# Autodesk Inventor assembly: Final Assembly
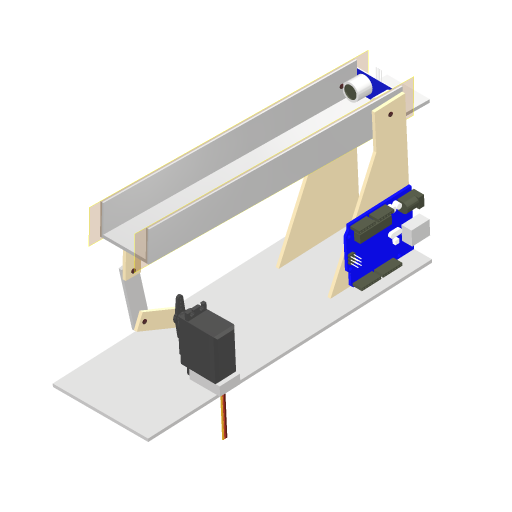
[picture p0: Inventor's stored thumbnail of the model, 512x512]
Saved by Autodesk Inventor 2024 (Build 280153000, 153)
## iProperties
Created: 2024-10-17
Part Number: Final Assembly
Document SubType Name: Assembly
Designer: ASUS
Author: ASUS
## Documents named in this file (13)
- D:\Control System\CAD parts & assembly 2\CAD parts & assembly\Final Assembly.iam
- D:\Control System\CAD parts & assembly 2\CAD parts & assembly\base.ipt
- D:\Control System\CAD parts & assembly 2\CAD parts & assembly\stand.ipt
- D:\Control System\CAD parts & assembly 2\CAD parts & assembly\beam rails.ipt
- D:\Control System\CAD parts & assembly 2\CAD parts & assembly\dummy bolt.ipt
- D:\Control System\CAD parts & assembly 2\CAD parts & assembly\beam base.ipt
- D:\Control System\CAD parts & assembly 2\CAD parts & assembly\beam revolute.ipt
- D:\Control System\CAD parts & assembly 2\CAD parts & assembly\lever.ipt
- D:\Control System\CAD parts & assembly 2\CAD parts & assembly\arm.ipt
- D:\Control System\CAD parts & assembly 2\CAD parts & assembly\ultrasonik sensor\ultrasonik sensor.ipt
- D:\Control System\CAD parts & assembly 2\CAD parts & assembly\Servo - MG 996R\Servo - MG 996R.ipt
- D:\Control System\CAD parts & assembly 2\CAD parts & assembly\motor support.ipt
- D:\Control System\CAD parts & assembly 2\CAD parts & assembly\arduino uno\arduino uno.ipt
## Components (19 placed, 12 different names)
1. base:1 — Mate:1, Mate:2, Mate:3, Mate:4, Mate:5, Flush:1, Mate:17, Mate:22
2. stand:1 — Mate:1, Mate:5, Flush:1, Mate:7, Insert:1
3. stand:2 — Mate:2, Mate:3, Mate:4, Mate:6, Insert:2, Mate:21, Flush:13
4. beam rails:1 — Mate:6, Insert:4, Mate:9, Flush:2, Flush:5, Mate:18
5. beam rails:2 — Mate:7, Insert:3, Mate:8, Flush:3, Flush:4, Flush:7, Mate:19, Mate:23
6. dummy bolt:1 — Insert:2, Insert:4
7. dummy bolt:2 — Insert:1, Insert:3
8. beam base:1 — Mate:8, Mate:9, Flush:2, Flush:3, Flush:4, Flush:5, Mate:10, Flush:6, Mate:20
9. beam revolute:1 — Mate:10, Flush:6, Flush:7, Insert:5, Mate:11
10. lever:1 — Insert:6, Mate:11, Mate:12, Insert:7
11. dummy bolt:3 — Insert:5, Insert:6
12. arm:1 — Mate:12, Insert:8
13. dummy bolt:4 — Insert:7, Insert:8
14. ultrasonik sensor:1 — Mate:18, Mate:19, Mate:20, Mate:23
15. Servo - MG 996R:1 — Mate:15, Mate:16, Flush:12
16. motor support:1 — Mate:13, Flush:9, Flush:11, Mate:15
17. motor support:2 — Mate:13, Mate:14, Flush:8, Flush:9, Flush:10, Flush:11, Mate:16, Flush:12
18. motor support:3 — Mate:14, Flush:8, Flush:10, Mate:17
19. arduino uno:1 — Mate:21, Flush:13, Mate:22
## Relationships (44: Mate 23, Flush 13, Insert 8)
- Mate:1: base:1 ↔ stand:1
- Mate:2: base:1 ↔ stand:2
- Mate:3: base:1 ↔ stand:2
- Mate:4: base:1 ↔ stand:2
- Mate:5: base:1 ↔ stand:1
- Flush:1: base:1 ↔ stand:1
- Mate:6: stand:2 ↔ beam rails:1
- Mate:7: stand:1 ↔ beam rails:2
- Insert:1 (-0.5 mm): stand:1 ↔ dummy bolt:2
- Insert:2 (-0.5 mm): stand:2 ↔ dummy bolt:1
- Insert:3 (-0.5 mm): beam rails:2 ↔ dummy bolt:2
- Insert:4 (-0.5 mm): beam rails:1 ↔ dummy bolt:1
- Mate:8: beam rails:2 ↔ beam base:1
- Mate:9: beam rails:1 ↔ beam base:1
- Flush:2: beam rails:1 ↔ beam base:1
- Flush:3: beam rails:2 ↔ beam base:1
- Flush:4: beam rails:2 ↔ beam base:1
- Flush:5: beam rails:1 ↔ beam base:1
- Mate:10: beam base:1 ↔ beam revolute:1
- Flush:6: beam base:1 ↔ beam revolute:1
- Flush:7 (22.5 mm): beam rails:2 ↔ beam revolute:1
- Insert:5 (-0.5 mm): beam revolute:1 ↔ dummy bolt:3
- Insert:6 (0.5 mm): lever:1 ↔ dummy bolt:3
- Mate:11: beam revolute:1 ↔ lever:1
- Mate:12: lever:1 ↔ arm:1
- Insert:7 (-0.5 mm): lever:1 ↔ dummy bolt:4
- Insert:8 (-0.5 mm): arm:1 ↔ dummy bolt:4
- Mate:13: motor support:1 ↔ motor support:2
- Mate:14: motor support:2 ↔ motor support:3
- Flush:8: motor support:2 ↔ motor support:3
- Flush:9: motor support:1 ↔ motor support:2
- Flush:10: motor support:2 ↔ motor support:3
- Flush:11: motor support:1 ↔ motor support:2
- Mate:15: Servo - MG 996R:1 ↔ motor support:1
- Mate:16: Servo - MG 996R:1 ↔ motor support:2
- Flush:12 (0.2 mm): Servo - MG 996R:1 ↔ motor support:2
- Mate:17: base:1 ↔ motor support:3
- Mate:18: beam rails:1 ↔ ultrasonik sensor:1
- Mate:19: beam rails:2 ↔ ultrasonik sensor:1
- Mate:20: beam base:1 ↔ ultrasonik sensor:1
- Mate:21: stand:2 ↔ arduino uno:1
- Flush:13: stand:2 ↔ arduino uno:1
- Mate:22: base:1 ↔ arduino uno:1
- Mate:23 (-1.6 mm): beam rails:2 ↔ ultrasonik sensor:1
## Named parameters: Finish1_Area = 587.617, Finish2_Area = 584.557, Finish3_Area = 285.786, Finish4_Area = 9.19867, Finish5_Area = 16.8487, Finish6_Area = 4.52389
note: some values were not read from the file. Shown as the stored number, unit unknown: "Finish1_Area", "Finish2_Area", "Finish3_Area", "Finish4_Area", "Finish5_Area", "Finish6_Area".
